# Autodesk Inventor assembly: BaseaSS
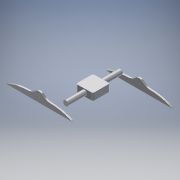
[picture p0: Inventor's stored thumbnail of the model, 180x180]
Saved by Autodesk Inventor 2016 (Build 200138000, 138)
## iProperties
Created: 2017-12-18
Part Number: BaseaSS
Document SubType Name: Assembly
Designer: student
Author: student
## Documents named in this file (4)
- C:\Users\student\Documents\GitHub\POV2017\INVENTOR\BaseaSS.iam
- C:\Users\student\Documents\GitHub\POV2017\INVENTOR\holder.ipt
- C:\Users\student\Documents\GitHub\POV2017\INVENTOR\Rod.ipt
- C:\Users\student\Documents\GitHub\POV2017\INVENTOR\basemotor.ipt
## Components (5 placed, 3 different names)
1. Rod:1 — Mate:1, Mate:2, Mate:6, Mate:8
2. basemotor:1 — Mate:1, Mate:2, Mate:3, Mate:4
3. Rod:2 — Mate:3, Mate:4
4. holder:1 — Mate:6, Mate:8
5. holder:2
## Relationships (6: Mate 6)
- Mate:1: Rod:1 ↔ basemotor:1
- Mate:2: Rod:1 ↔ basemotor:1
- Mate:3: basemotor:1 ↔ Rod:2
- Mate:4: basemotor:1 ↔ Rod:2
- Mate:6: Rod:1 ↔ holder:1
- Mate:8: Rod:1 ↔ holder:1
